# Autodesk Inventor assembly: hv
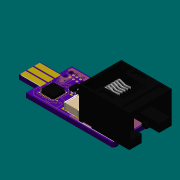
[picture p0: Inventor's stored thumbnail of the model, 180x180]
Saved by Autodesk Inventor 2016 (Build 200138000, 138)
## iProperties
Created: 2015-11-05
Part Number: hv
Document SubType Name: Assembly
Designer: Sawaiz
Author: Sawaiz
## Documents named in this file (14)
- C:\Users\Sawaiz\OneDrive\projects\mppcSensorInterface\cad\hvBoard\hv.iam
- C:\Users\Sawaiz\OneDrive\projects\mppcSensorInterface\cad\hvBoard\pcb.ipt
- C:\Users\Sawaiz\OneDrive\projects\mppcSensorInterface\cad\electronics\chipResistor\chipResistor-0402.ipt
- C:\Users\Sawaiz\OneDrive\projects\mppcSensorInterface\cad\electronics\chipResistor.ipt
- C:\Users\Sawaiz\OneDrive\projects\mppcSensorInterface\cad\electronics\capacitor-0402.ipt
- C:\Users\Sawaiz\OneDrive\projects\mppcSensorInterface\cad\electronics\capacitor.ipt
- C:\Users\Sawaiz\OneDrive\projects\mppcSensorInterface\cad\electronics\qfnEven\qfnEven-32.ipt
- C:\Users\Sawaiz\OneDrive\projects\mppcSensorInterface\cad\electronics\qfnEven.ipt
- C:\Users\Sawaiz\OneDrive\projects\mppcSensorInterface\cad\electronics\SOT23-3.ipt
- C:\Users\Sawaiz\OneDrive\projects\mppcSensorInterface\cad\capacitor-2220.ipt
- C:\Users\Sawaiz\OneDrive\projects\mppcSensorInterface\cad\electronics\SDR0503.ipt
- C:\Users\Sawaiz\OneDrive\projects\mppcSensorInterface\cad\electronics\import\MOLEX_0955012882.ipt
- C:\Users\Sawaiz\OneDrive\projects\mppcSensorInterface\cad\electronics\sod-80.ipt
- C:\Users\Sawaiz\OneDrive\projects\mppcSensorInterface\cad\electronics\S3O8.ipt
## Components (13 placed, 10 different names)
1. pcb:1 — Angle:1, Tangent:1, Mate:1, Flush:10, Mate:2, Angle:11
2. chipResistor-0402:1 — Flush:3, Flush:4, Angle:2, Angle:3
3. chipResistor-0402:2 — Flush:2, Flush:3, Angle:5, Flush:6, Angle:7, Angle:8, Angle:9, Flush:8
4. capacitor-0402:1 — Flush:1, Flush:2, Angle:4, Angle:5, Angle:6
5. capacitor-0402:2 — Flush:1, Angle:3, Angle:4
6. qfnEven-32:1 — Flush:4, Angle:1, Angle:2, Flush:7
7. SOT23-3:1 — Flush:5, Angle:7
8. SOT23-3:2 — Flush:5, Flush:6, Angle:6
9. capacitor-2220:3 — Flush:7, Angle:8, Angle:10, Mate:1
10. SDR0503:1 — Angle:9, Flush:8, Flush:9
11. MOLEX_0955012882:1 — Flush:9, Angle:10, Flush:10
12. sod-80:1 — Tangent:1
13. S3O8:1 — Mate:2, Angle:11
## Relationships (24: Angle 11, Flush 10, Mate 2, Tangent 1)
- Flush:1: capacitor-0402:1 ↔ capacitor-0402:2
- Flush:2: chipResistor-0402:2 ↔ capacitor-0402:1
- Flush:3: chipResistor-0402:1 ↔ chipResistor-0402:2
- Flush:4: chipResistor-0402:1 ↔ qfnEven-32:1
- Angle:1 (0 deg): pcb:1 ↔ qfnEven-32:1
- Angle:2 (0 deg): chipResistor-0402:1 ↔ qfnEven-32:1
- Angle:3 (0 deg): chipResistor-0402:1 ↔ capacitor-0402:2
- Angle:4 (0 deg): capacitor-0402:1 ↔ capacitor-0402:2
- Angle:5 (0 deg): chipResistor-0402:2 ↔ capacitor-0402:1
- Flush:5: SOT23-3:1 ↔ SOT23-3:2
- Flush:6: chipResistor-0402:2 ↔ SOT23-3:2
- Angle:6 (0 deg): capacitor-0402:1 ↔ SOT23-3:2
- Angle:7 (0 deg): chipResistor-0402:2 ↔ SOT23-3:1
- Flush:7: qfnEven-32:1 ↔ capacitor-2220:3
- Angle:8 (0 deg): chipResistor-0402:2 ↔ capacitor-2220:3
- Angle:9 (0 deg): chipResistor-0402:2 ↔ SDR0503:1
- Flush:8: chipResistor-0402:2 ↔ SDR0503:1
- Flush:9: SDR0503:1 ↔ MOLEX_0955012882:1
- Angle:10 (0 deg): capacitor-2220:3 ↔ MOLEX_0955012882:1
- Tangent:1: pcb:1 ↔ sod-80:1
- Mate:1: pcb:1 ↔ capacitor-2220:3
- Flush:10 (0.5953 mm): pcb:1 ↔ MOLEX_0955012882:1
- Mate:2: pcb:1 ↔ S3O8:1
- Angle:11 (0 deg): pcb:1 ↔ S3O8:1
